# Autodesk Inventor assembly: PlanetaryGear
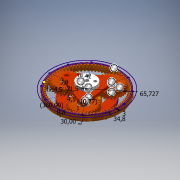
[picture p0: Inventor's stored thumbnail of the model, 180x180]
Saved by Autodesk Inventor 2018.3 (Build 223284000, 284)
## iProperties
Created: 2018-07-08
Part Number: PlanetaryGear
Material: Generisch
Document SubType Name: Assembly
Designer: JochenAlt
Author: JochenAlt
## Documents named in this file (9)
- D:\Projects\FlowerPot\CAD\PlanetaryGear\PlanetaryGear.iam
- D:\Projects\FlowerPot\CAD\PlanetaryGear\Konstruktions-Assistent\Stirnzahnrad21.ipt
- D:\Projects\FlowerPot\CAD\PlanetaryGear\Konstruktions-Assistent\Stirnzahnrad23.ipt
- D:\Projects\FlowerPot\CAD\PlanetaryGear\PlanetaryHolder.ipt
- D:\Projects\FlowerPot\CAD\PlanetaryGear\PlanetaryHolderTop.ipt
- D:\Projects\FlowerPot\CAD\Mounting Hub.ipt
- D:\Projects\FlowerPot\CAD\PlanetaryGear\PlanetaryHolderBottom.ipt
- D:\Projects\FlowerPot\CAD\PlanetaryGear\PlanetaryGearConstr\Konstruktions-Assistent\Stirnzahnrad12.ipt
- C:\Users\JochenAlt\Documents\Inventor\Content Center Files\R2018\de-DE\DIN BEARING(1)\DIN 625 SKF - SKF 623.ipt
## Components (12 placed, 7 different names)
1. Stirnzahnrad2:1 — Fluchtend:1, Passend:13, Drehung:3, Drehung:4
2. Stirnzahnrad2:2 — Fluchtend:1, Fluchtend:4, Fluchtend:5, Passend:16, Passend:19, Drehung:9
3. Stirnzahnrad2:3 — Fluchtend:3, Passend:18, Passend:21, Drehung:3, Passend:29, Drehung:6
4. Stirnzahnrad2:4 — Fluchtend:2, Fluchtend:6, Passend:17, Passend:20, Drehung:4, Drehung:7
5. PlanetaryHolder:1
6. PlanetaryHolderTop:1 — Passend:1, Passend:2, Passend:26, Passend:27, Passend:28, Passend:29
7. Mounting Hub:1 — Passend:1, Passend:2
8. PlanetaryHolderBottom:1 — Passend:15, Passend:16, Passend:17, Passend:18, Passend:23, Passend:24, Passend:25, Passend:26, Passend:27, Passend:28, Drehung:5
9. Stirnzahnrad1:1 — Fluchtend:2, Passend:14, Fluchtend:3, Fluchtend:4, Fluchtend:5, Fluchtend:6, Drehung:5, Drehung:6, Drehung:7, Drehung:8, Drehung:9
10. DIN 625 SKF SKF 623:1 — Passend:19, Passend:23, Drehung:8
11. DIN 625 SKF SKF 623:2 — Passend:20, Passend:24
12. DIN 625 SKF SKF 623:3 — Passend:21, Passend:25
## Relationships (31: Mate 18, RelateRotation 7, Flush 6)
- Passend:1 [Mate]: PlanetaryHolderTop:1 ↔ Mounting Hub:1
- Passend:2 [Mate]: PlanetaryHolderTop:1 ↔ Mounting Hub:1
- Fluchtend:1 [Flush]: Stirnzahnrad2:1 ↔ Stirnzahnrad2:2
- Fluchtend:2 [Flush]: Stirnzahnrad2:4 ↔ Stirnzahnrad1:1
- Passend:13 [Mate]: Stirnzahnrad2:1
- Passend:14 [Mate]: Stirnzahnrad1:1
- Passend:15 [Mate]: PlanetaryHolderBottom:1
- Fluchtend:3 [Flush]: Stirnzahnrad2:3 ↔ Stirnzahnrad1:1
- Fluchtend:4 [Flush]: Stirnzahnrad2:2 ↔ Stirnzahnrad1:1
- Fluchtend:5 [Flush]: Stirnzahnrad2:2 ↔ Stirnzahnrad1:1
- Fluchtend:6 [Flush]: Stirnzahnrad2:4 ↔ Stirnzahnrad1:1
- Passend:16 [Mate]: Stirnzahnrad2:2 ↔ PlanetaryHolderBottom:1
- Passend:17 [Mate]: Stirnzahnrad2:4 ↔ PlanetaryHolderBottom:1
- Passend:18 [Mate]: Stirnzahnrad2:3 ↔ PlanetaryHolderBottom:1
- Passend:19 [Mate]: Stirnzahnrad2:2 ↔ DIN 625 SKF SKF 623:1
- Passend:20 [Mate]: Stirnzahnrad2:4 ↔ DIN 625 SKF SKF 623:2
- Passend:21 [Mate]: Stirnzahnrad2:3 ↔ DIN 625 SKF SKF 623:3
- Passend:23 [Mate]: PlanetaryHolderBottom:1 ↔ DIN 625 SKF SKF 623:1
- Passend:24 [Mate]: PlanetaryHolderBottom:1 ↔ DIN 625 SKF SKF 623:2
- Passend:25 [Mate]: PlanetaryHolderBottom:1 ↔ DIN 625 SKF SKF 623:3
- Passend:26 [Mate]: PlanetaryHolderTop:1 ↔ PlanetaryHolderBottom:1
- Passend:27 [Mate]: PlanetaryHolderTop:1 ↔ PlanetaryHolderBottom:1
- Passend:28 [Mate]: PlanetaryHolderTop:1 ↔ PlanetaryHolderBottom:1
- Drehung:3 [RelateRotation] (-0.4 ul): Stirnzahnrad2:1 ↔ Stirnzahnrad2:3
- Drehung:4 [RelateRotation] (-0.4 ul): Stirnzahnrad2:1 ↔ Stirnzahnrad2:4
- Drehung:5 [RelateRotation] (-0.2 ul): PlanetaryHolderBottom:1 ↔ Stirnzahnrad1:1
- Passend:29 [Mate] (1 mm): Stirnzahnrad2:3 ↔ PlanetaryHolderTop:1
- Drehung:6 [RelateRotation] (-0.3 ul): Stirnzahnrad2:3 ↔ Stirnzahnrad1:1
- Drehung:7 [RelateRotation] (-0.3 ul): Stirnzahnrad2:4 ↔ Stirnzahnrad1:1
- Drehung:8 [RelateRotation] (0.3 ul): Stirnzahnrad1:1 ↔ DIN 625 SKF SKF 623:1
- Drehung:9 [RelateRotation] (0.3 ul): Stirnzahnrad2:2 ↔ Stirnzahnrad1:1
